# Autodesk Inventor assembly: Side Panel
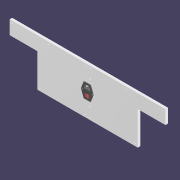
[picture p0: Inventor's stored thumbnail of the model, 180x180]
Saved by Autodesk Inventor 2017 SP1 (Build 210196100, 196)
## iProperties
Created: 2017-08-09
Part Number: Side Panel
Document SubType Name: Assembly
Designer: Zach
Mass: 1082.83 g
Surface Area: 2492.77 cm^2
Volume: 1022.19 cm^3
Density: 1.05932 g/cm^3
Author: Zach
## Documents named in this file (4)
- C:\Users\Zach\Documents\GitHub\tr1\src\Base\Side Panel\Side Panel Back.iam
- C:\Users\Zach\Documents\GitHub\tr1\lib\Power Switch\Power Switch.iam
- C:\Users\Zach\Documents\GitHub\tr1\src\Base\Side Panel\SP005b.ipt
- C:\Users\Zach\Documents\GitHub\tr1\src\Base\Side Panel\SP006b.ipt
## Components (3 placed, 3 different names)
1. Power Switch:1 [sub-assembly] — Mate:45, Mate:46, Mate:47
2. SP005b:1 — Mate:42, Mate:43, Mate:44, Mate:45, Mate:46, Mate:47
3. SP006b:1 — Mate:42, Mate:43, Mate:44
## Relationships (6: Mate 6)
- Mate:42: SP005b:1 ↔ SP006b:1
- Mate:43: SP005b:1 ↔ SP006b:1
- Mate:44: SP005b:1 ↔ SP006b:1
- Mate:45: Power Switch:1 ↔ SP005b:1
- Mate:46: Power Switch:1 ↔ SP005b:1
- Mate:47: Power Switch:1 ↔ SP005b:1
